# Autodesk Inventor assembly: ensambleparlante
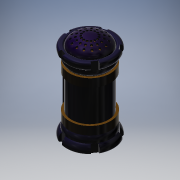
[picture p0: Inventor's stored thumbnail of the model, 180x180]
Saved by Autodesk Inventor 2019 (Build 230136000, 136)
## iProperties
Created: 2019-03-07
Part Number: ensambleparlante
Material: Genérico
Document SubType Name: Assembly
Designer: flakt
Author: flakt
## Documents named in this file (3)
- D:\Documents\Kevin\robot\ensambleparlante.iam
- D:\Documents\Kevin\robot\caseparlante.ipt
- D:\Documents\Kevin\robot\tapaparlante.ipt
## Components (3 placed, 2 different names)
1. caseparlante:1 — De rotación:1, De rotación:2
2. tapaparlante:1 — De rotación:1
3. tapaparlante:2 — De rotación:2
## Relationships (2: RevoluteJoint 2)
- De rotación:1 [RevoluteJoint] (6 mm): caseparlante:1 ↔ tapaparlante:1
- De rotación:2 [RevoluteJoint] (6 mm): caseparlante:1 ↔ tapaparlante:2
